# Autodesk Inventor assembly: Battery Bank 3x14 Rear A
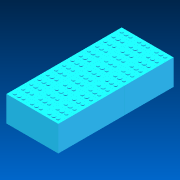
[picture p0: Inventor's stored thumbnail of the model, 180x180]
Saved by Autodesk Inventor 2012 (Build 160160000, 160)
## iProperties
Created: 2012-07-01
Part Number: Battery Bank 3x14 Rear A
Document SubType Name: Assembly
Designer: Hemant
Author: Hemant
## Documents named in this file (2)
- C:\Users\Hemant\Documents\Pastic Box - Rear A\Battery Bank 3x14 Rear A.iam
- C:\Users\Hemant\Documents\CALB100AH.ipt
## Components (42 placed, 1 different names)
1. CALB100AH:1
2. CALB100AH:2
3. CALB100AH:3
4. CALB100AH:4
5. CALB100AH:5
6. CALB100AH:6
7. CALB100AH:7
8. CALB100AH:8
9. CALB100AH:9
10. CALB100AH:10
11. CALB100AH:11
12. CALB100AH:12
13. CALB100AH:13
14. CALB100AH:14
15. CALB100AH:15
16. CALB100AH:16
17. CALB100AH:17
18. CALB100AH:18
19. CALB100AH:19
20. CALB100AH:20
21. CALB100AH:21
22. CALB100AH:22
23. CALB100AH:23
24. CALB100AH:24
25. CALB100AH:25
26. CALB100AH:26
27. CALB100AH:27
28. CALB100AH:28
29. CALB100AH:29
30. CALB100AH:30
31. CALB100AH:31
32. CALB100AH:32
33. CALB100AH:33
34. CALB100AH:34
35. CALB100AH:35
36. CALB100AH:36
37. CALB100AH:37
38. CALB100AH:38
39. CALB100AH:39
40. CALB100AH:40
41. CALB100AH:41
42. CALB100AH:42
## Component patterns: (42 elements, first: CALB100AH:1)
